# Autodesk Inventor assembly: Ruedas de soporte
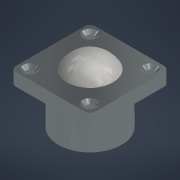
[picture p0: Inventor's stored thumbnail of the model, 180x180]
Saved by Autodesk Inventor 2022 (Build 260153000, 153)
## iProperties
Part Number: Ruedas de soporte
Document SubType Name: Ensamblaje
Designer: seb_0
Author: seb_0
## Documents named in this file (3)
- D:\Documentos\15.PUCP_2021-2\[PDM] Proyecto de Diseño Mecatrónico\ProyectoGIT\ProyectoRobotPallet\RuedasAuxiliares\Ruedas de soporte.iam
- D:\Documentos\15.PUCP_2021-2\[PDM] Proyecto de Diseño Mecatrónico\ProyectoGIT\ProyectoRobotPallet\RuedasAuxiliares\Soporte.ipt
- D:\Documentos\15.PUCP_2021-2\[PDM] Proyecto de Diseño Mecatrónico\ProyectoGIT\ProyectoRobotPallet\RuedasAuxiliares\Rueda.ipt
## Components (2 placed, 2 different names)
1. Soporte:1 — Coincidencia:1, Coincidencia:2, Coincidencia:3, Coincidencia:4
2. Rueda:1 — Coincidencia:1
## Relationships (4: Mate 4)
- Coincidencia:1 [Mate]: Soporte:1 ↔ Rueda:1
- Coincidencia:2 [Mate]: Soporte:1
- Coincidencia:3 [Mate]: Soporte:1
- Coincidencia:4 [Mate] (12.94 mm): Soporte:1
